# Autodesk Inventor assembly: шутер
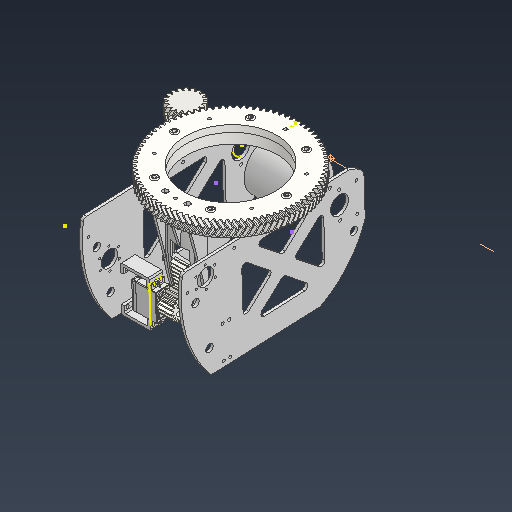
[picture p0: Inventor's stored thumbnail of the model, 512x512]
Saved by Autodesk Inventor 2026 (Build 300175000, 175)
## iProperties
Created: 2026-01-10
Part Number: шутер
Document SubType Name: Assembly
Designer: GameHD
Author: GameHD
## Documents named in this file (12)
- C:\Users\GameHD\Desktop\Phantom 16950\шутер.iam
- C:\Users\GameHD\Desktop\Phantom 16950\стенка пуляло.ipt
- C:\Users\GameHD\Desktop\Phantom 16950\шевронное очко.iam
- C:\Users\GameHD\Desktop\Phantom 16950\шестерня стрелять\шестерня стрелять\шестерня стрелять.ipt
- C:\Users\GameHD\Desktop\Phantom 16950\изгиб новый.ipt
- C:\Users\GameHD\Desktop\Phantom 16950\СИСЬКА.ipt
- C:\Users\GameHD\Desktop\Phantom 16950\угол 25-26_MIR_MIR.ipt
- C:\Users\GameHD\Desktop\Phantom 16950\серва мотор.ipt
- C:\Users\GameHD\Desktop\Phantom 16950\шестерни прямые изменяемая траектория.iam
- C:\Users\GameHD\Desktop\Phantom 16950\крепл сервы на пуляло.ipt
- C:\Users\GameHD\Downloads\Telegram Desktop\шестерня прям мал для траектории (2)\шестерня прям мал для траектории (2)\шестерня прям мал для траектории (2).ipt
- C:\Users\GameHD\Desktop\Phantom 16950\стенка пуляло ответная.ipt
## Components (13 placed, 11 different names)
1. стенка пуляло:1 — Совмещение:5, Совмещение:6, Совмещение:8, Совмещение:9, Совмещение:14, Совмещение:15, Совмещение:16, Совмещение:17, Совмещение:20, Совмещение:26, Совмещение:27
2. шевронное очко:1 [sub-assembly]
3. шестерня стрелять:1 — Совмещение:5, Совмещение:7, Совмещение:31, Совмещение:32
4. изгиб новый:1 — Заподлицо:2, Совмещение:10, Совмещение:25
5. СИСЬКА:1 — Совмещение:6, Заподлицо:2
6. угол 25-26_MIR_MIR:1 — Совмещение:7, Совмещение:8, Совмещение:9
7. серва мотор:1 — Совмещение:18, Совмещение:19, Совмещение:21, Совмещение:22, Совмещение:23, Совмещение:24
8. шестерни прямые изменяемая траектория:1 [sub-assembly] — Совмещение:10, Совмещение:25, ЗубчПер:1
9. крепл сервы на пуляло:1 — Совмещение:14, Совмещение:16, Совмещение:17, Заподлицо:3, Совмещение:18, Совмещение:19
10. крепл сервы на пуляло:2 — Совмещение:15, Заподлицо:3, Совмещение:20, Совмещение:21, Совмещение:23
11. шестерня прям мал для траектории (2):1 — Совмещение:22, Совмещение:24, ЗубчПер:1
12. стенка пуляло ответная:1 — Совмещение:26, Совмещение:27, Совмещение:30
13. угол 25-26_MIR_MIR:2 — Совмещение:30, Совмещение:31, Совмещение:32
## Relationships (31: Mate 27, Flush 3, RelateRotation 1)
- [Flush]: шевронное очко:1 ↔ шестерня стрелять:1
- [Mate]: шевронное очко:1 ↔ шестерня стрелять:1
- [Mate]: шестерня стрелять:1 ↔ изгиб новый:1
- [Mate]: шестерня стрелять:1 ↔ изгиб новый:1
- [Mate]: шестерня стрелять:1 ↔ изгиб новый:1
- Совмещение:5 [Mate]: стенка пуляло:1 ↔ шестерня стрелять:1
- Совмещение:6 [Mate]: стенка пуляло:1 ↔ СИСЬКА:1
- Совмещение:7 [Mate]: шестерня стрелять:1 ↔ угол 25-26_MIR_MIR:1
- Совмещение:8 [Mate]: стенка пуляло:1 ↔ угол 25-26_MIR_MIR:1
- Совмещение:9 [Mate]: стенка пуляло:1 ↔ угол 25-26_MIR_MIR:1
- Заподлицо:2 [Flush]: изгиб новый:1 ↔ СИСЬКА:1
- Совмещение:10 [Mate]: изгиб новый:1 ↔ шестерни прямые изменяемая траектория:1
- Совмещение:14 [Mate]: стенка пуляло:1 ↔ крепл сервы на пуляло:1
- Совмещение:15 [Mate]: стенка пуляло:1 ↔ крепл сервы на пуляло:2
- Совмещение:16 [Mate]: стенка пуляло:1 ↔ крепл сервы на пуляло:1
- Совмещение:17 [Mate]: стенка пуляло:1 ↔ крепл сервы на пуляло:1
- Заподлицо:3 [Flush]: крепл сервы на пуляло:1 ↔ крепл сервы на пуляло:2
- Совмещение:18 [Mate]: серва мотор:1 ↔ крепл сервы на пуляло:1
- Совмещение:19 [Mate]: серва мотор:1 ↔ крепл сервы на пуляло:1
- Совмещение:20 [Mate]: стенка пуляло:1 ↔ крепл сервы на пуляло:2
- Совмещение:21 [Mate]: серва мотор:1 ↔ крепл сервы на пуляло:2
- Совмещение:22 [Mate] (3.5 mm): серва мотор:1 ↔ шестерня прям мал для траектории (2):1
- Совмещение:23 [Mate]: серва мотор:1 ↔ крепл сервы на пуляло:2
- Совмещение:24 [Mate]: серва мотор:1 ↔ шестерня прям мал для траектории (2):1
- Совмещение:25 [Mate]: изгиб новый:1 ↔ шестерни прямые изменяемая траектория:1
- ЗубчПер:1 [RelateRotation] (0.933 ul): шестерни прямые изменяемая траектория:1 ↔ шестерня прям мал для траектории (2):1
- Совмещение:26 [Mate]: стенка пуляло:1 ↔ стенка пуляло ответная:1
- Совмещение:27 [Mate]: стенка пуляло:1 ↔ стенка пуляло ответная:1
- Совмещение:30 [Mate]: стенка пуляло ответная:1 ↔ угол 25-26_MIR_MIR:2
- Совмещение:31 [Mate]: шестерня стрелять:1 ↔ угол 25-26_MIR_MIR:2
- Совмещение:32 [Mate]: шестерня стрелять:1 ↔ угол 25-26_MIR_MIR:2
